# Autodesk Inventor assembly: rev2 full
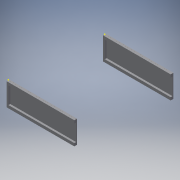
[picture p0: Inventor's stored thumbnail of the model, 180x180]
Saved by Autodesk Inventor 2017 (Build 210142000, 142)
## iProperties
Created: 2019-05-04
Part Number: rev2 full
Document SubType Name: Assembly
Designer: Roman
Author: Roman
## Documents named in this file (2)
- C:\Users\Roman\Documents\CAD\enclosure rev1\rev2 full.iam
- C:\Users\Roman\Documents\CAD\enclosure rev1\rev2 base\rev1 large wall\rev1 base large wall.iam
## Components (2 placed, 1 different names)
1. rev1 base large wall:1 [sub-assembly]
2. rev1 base large wall:2 [sub-assembly]
## Named parameters: height = 25.4 mm
